# Autodesk Inventor assembly: TP-Link_bodo
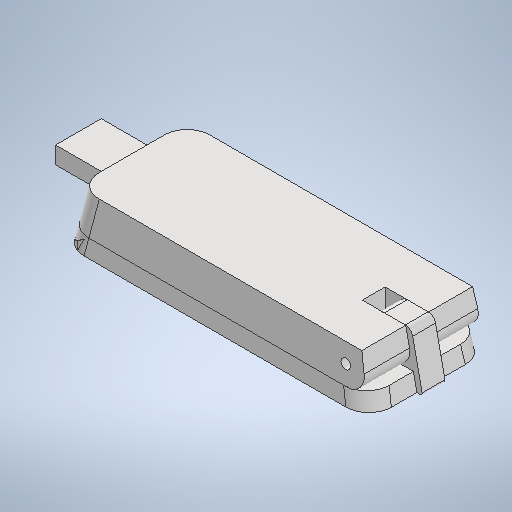
[picture p0: Inventor's stored thumbnail of the model, 512x512]
Saved by Autodesk Inventor 2025.1 (Build 291241000, 241)
## iProperties
Created: 2026-04-16
Part Number: TP-Link_bodo
Document SubType Name: Assembly
Designer: User
Author: User
## Documents named in this file (3)
- D:\One Drive\OneDrive - Politeknik Sultan Salahuddin Abdul Aziz Shah\Documents\Inventor\RobosotPSA\TP-Link_bodo.iam
- D:\One Drive\OneDrive - Politeknik Sultan Salahuddin Abdul Aziz Shah\Documents\Inventor\RobosotPSA\ArcherT4U_USB.ipt
- D:\One Drive\OneDrive - Politeknik Sultan Salahuddin Abdul Aziz Shah\Documents\Inventor\RobosotPSA\ArcherT4U_Antena.ipt
## Components (2 placed, 2 different names)
1. ArcherT4U_USB:1 — Flush:1
2. ArcherT4U_Antena:1 — Flush:1
## Relationships (1: Flush 1)
- Flush:1: ArcherT4U_USB:1 ↔ ArcherT4U_Antena:1
